# Autodesk Inventor assembly: MAQUINADO CAVIDAD 2 CLASE
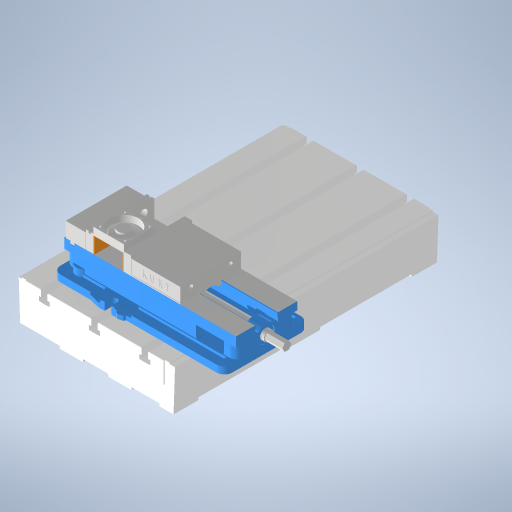
[picture p0: Inventor's stored thumbnail of the model, 512x512]
Saved by Autodesk Inventor 2023.2 (Build 272271030, 271C)
## iProperties
Created: 2023-08-14
Part Number: MAQUINADO CAVIDAD 2 CLASE
Document SubType Name: Assembly
Designer: Cris Pat
Sending System: Autodesk Inventor 2024
Preprocessor: ST-DEVELOPER v19.2
Title: 7 - MAQUINADO CAVIDAD 2 (VACO).stp
Author: ARViau
## Documents named in this file (4)
- C:\Users\Cris Pat\Desktop\U\Semestre_10\Disenio_y_manufactura\feature_zip\7 - MAQUINADO CAVIDAD 2 (VACÍO)\7 - MAQUINADO CAVIDAD 2 (VACÍO).iam
- C:\Users\Cris Pat\Desktop\U\Semestre_10\Disenio_y_manufactura\feature_zip\VF1 TABLE + FLEX_KURT D688.iam
- C:\Users\Cris Pat\Desktop\U\Semestre_10\Disenio_y_manufactura\feature_zip\6 - CAVIDAD MATERIAL 2.ipt
- C:\Users\Cris Pat\Desktop\U\Semestre_10\Disenio_y_manufactura\feature_zip\ALZA MAQUINADO.ipt
## Components (4 placed, 3 different names)
1. VF1 TABLE + FLEX_KURT D688:1 [sub-assembly] — Mate:1, Flush:1, Mate:2, Mate:3, Mate:4, Flush:2, Flush:3, Mate:6
2. 6 - CAVIDAD MATERIAL 2:1 — Mate:5, Flush:3, Mate:6
3. ALZA MAQUINADO:1 — Mate:1, Flush:1, Mate:2
4. ALZA MAQUINADO:2 — Mate:3, Mate:4, Flush:2, Mate:5
## Relationships (9: Mate 6, Flush 3)
- Mate:1: VF1 TABLE + FLEX_KURT D688:1 ↔ ALZA MAQUINADO:1
- Flush:1: VF1 TABLE + FLEX_KURT D688:1 ↔ ALZA MAQUINADO:1
- Mate:2: VF1 TABLE + FLEX_KURT D688:1 ↔ ALZA MAQUINADO:1
- Mate:3: VF1 TABLE + FLEX_KURT D688:1 ↔ ALZA MAQUINADO:2
- Mate:4: VF1 TABLE + FLEX_KURT D688:1 ↔ ALZA MAQUINADO:2
- Flush:2: VF1 TABLE + FLEX_KURT D688:1 ↔ ALZA MAQUINADO:2
- Mate:5: 6 - CAVIDAD MATERIAL 2:1 ↔ ALZA MAQUINADO:2
- Flush:3: VF1 TABLE + FLEX_KURT D688:1 ↔ 6 - CAVIDAD MATERIAL 2:1
- Mate:6: VF1 TABLE + FLEX_KURT D688:1 ↔ 6 - CAVIDAD MATERIAL 2:1
